# Autodesk Inventor assembly: HbSocketU02
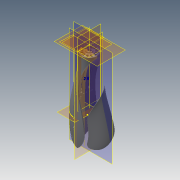
[picture p0: Inventor's stored thumbnail of the model, 180x180]
Saved by Autodesk Inventor 2015 SP1 (Build 190203100, 203)
## iProperties
Created: 2015-02-09
Part Number: HbSocketU02
Document SubType Name: Assembly
Designer: Yamaura
Author: Yamaura
## Documents named in this file (17)
- C:\Users\Yamaura\Documents\GitHub\HACKberry\HACKberry-hardware\3D\Inventor\Parts\HbSocketU02.iam
- C:\Users\Yamaura\Documents\GitHub\HACKberry\HACKberry-hardware\3D\Inventor\Parts\HbBatteryDoor03.ipt
- C:\Users\Yamaura\Documents\GitHub\HACKberry\HACKberry-hardware\3D\Inventor\Parts\HbBatteryDoorKnob03.ipt
- C:\Users\Yamaura\Documents\GitHub\HACKberry\HACKberry-hardware\3D\Inventor\Parts\HbBatteryHingeA03.ipt
- C:\Users\Yamaura\Documents\GitHub\HACKberry\HACKberry-hardware\3D\Inventor\Parts\HbBatteryHingeB03.ipt
- C:\Users\Yamaura\Documents\GitHub\HACKberry\HACKberry-hardware\3D\Inventor\Parts\HbBatteryHingeC03.ipt
- C:\Users\Yamaura\Documents\GitHub\HACKberry\HACKberry-hardware\3D\Inventor\Parts\HbBatteryCase01.ipt
- C:\Users\Yamaura\Documents\GitHub\HACKberry\HACKberry-hardware\3D\Inventor\Parts\HbBatteryLockKnob01.ipt
- C:\Users\Yamaura\Documents\GitHub\HACKberry\HACKberry-hardware\3D\Inventor\Parts\HbBatteryPcb01.ipt
- C:\Users\Yamaura\Documents\GitHub\HACKberry\HACKberry-hardware\3D\Inventor\Parts\DMW-BLF19.ipt
- C:\Users\Yamaura\Documents\GitHub\HACKberry\HACKberry-hardware\3D\Inventor\Parts\HbBatteryDoorLever03.ipt
- C:\Users\Yamaura\Documents\GitHub\HACKberry\HACKberry-hardware\3D\Inventor\Parts\HbMainFrameA01.ipt
- C:\Users\Yamaura\Documents\GitHub\HACKberry\HACKberry-hardware\3D\Inventor\Parts\HbMainFrameB01.ipt
- C:\Users\Yamaura\Documents\GitHub\HACKberry\HACKberry-hardware\3D\Inventor\Parts\HbUpperArmCover01.ipt
- C:\Users\Yamaura\Documents\GitHub\HACKberry\HACKberry-hardware\3D\Inventor\Parts\VN-3-1.ipt
- C:\Users\Yamaura\Documents\GitHub\HACKberry\HACKberry-hardware\3D\Inventor\Parts\TS 0.4-3.2-14.ipt
- C:\Users\Yamaura\Documents\GitHub\HACKberry\HACKberry-hardware\3D\Inventor\Parts\flatScrewM2L6PHI3.3T1.3.ipt
## Components (23 placed, 16 different names)
1. HbBatteryCase01:1 — メイト:29, メイト:30, メイト:34, メイト:35, メイト:36, フラッシュ:10, フラッシュ:11, フラッシュ:12, フラッシュ:13
2. HbBatteryLockKnob01:1 — メイト:30
3. HbBatteryPcb01:1 — メイト:29, メイト:61, メイト:62, メイト:63, メイト:64, メイト:69
4. DMW-BLF19:1 — メイト:34, メイト:35, メイト:36
5. flatScrewM2L6PHI3.3T1.3:1 — メイト:69, フラッシュ:10
6. flatScrewM2L6PHI3.3T1.3:2 — メイト:70, フラッシュ:12
7. flatScrewM2L6PHI3.3T1.3:3 — メイト:71, フラッシュ:13
8. flatScrewM2L6PHI3.3T1.3:4 — メイト:72, フラッシュ:11
9. TS 0.4-3.2-14:1 — メイト:73, 正接:1, 正接:2, 正接:3
10. VN-3-1:2 — メイト:62, メイト:63
11. HbBatteryHingeC03:1 — メイト:49, メイト:50, メイト:51
12. HbBatteryHingeB03:1 — メイト:40, メイト:45, メイト:47
13. HbBatteryHingeA03:1 — メイト:44, メイト:46
14. HbBatteryDoor03:1 — フラッシュ:5, メイト:44, メイト:45, メイト:46, メイト:47, メイト:49, メイト:50, メイト:51, 角度:3
15. HbMainFrameA01:1 — フラッシュ:6, フラッシュ:7, フラッシュ:8, メイト:52, メイト:53, メイト:54, メイト:73, 正接:1, 正接:2
16. VN-3-1:1 — メイト:61, メイト:64
17. HbBatteryDoorKnob03:3 — メイト:58, メイト:59, メイト:60, 正接:3
18. HbUpperArmCover01:1 — メイト:55, フラッシュ:9
19. HbMainFrameB01:1 — メイト:52, メイト:53, メイト:54, メイト:70, メイト:71, メイト:72
20. HbBatteryDoorKnob03:1 — メイト:37, メイト:38, メイト:39
21. HbBatteryDoorKnob03:2
22. HbBatteryDoorLever03:1 — メイト:37, メイト:38, メイト:39, メイト:58, メイト:59, メイト:60
23. HbBatteryDoorLever03:2
## Component patterns: (2 elements, first: HbBatteryDoorKnob03:1), (2 elements, first: HbBatteryDoorLever03:1)
## Relationships (45: Mate 32, Flush 9, Tangent 3, Angle 1)
- メイト:29 [Mate]: HbBatteryCase01:1 ↔ HbBatteryPcb01:1
- メイト:30 [Mate]: HbBatteryCase01:1 ↔ HbBatteryLockKnob01:1
- メイト:34 [Mate]: HbBatteryCase01:1 ↔ DMW-BLF19:1
- メイト:35 [Mate]: HbBatteryCase01:1 ↔ DMW-BLF19:1
- メイト:36 [Mate] (0.1 mm): HbBatteryCase01:1 ↔ DMW-BLF19:1
- メイト:37 [Mate]: HbBatteryDoorKnob03:1 ↔ HbBatteryDoorLever03:1
- メイト:38 [Mate]: HbBatteryDoorKnob03:1 ↔ HbBatteryDoorLever03:1
- メイト:39 [Mate]: HbBatteryDoorKnob03:1 ↔ HbBatteryDoorLever03:1
- メイト:40 [Mate]: HbBatteryHingeB03:1
- フラッシュ:5 [Flush]: HbBatteryDoor03:1
- メイト:44 [Mate]: HbBatteryHingeA03:1 ↔ HbBatteryDoor03:1
- メイト:45 [Mate]: HbBatteryHingeB03:1 ↔ HbBatteryDoor03:1
- メイト:46 [Mate]: HbBatteryHingeA03:1 ↔ HbBatteryDoor03:1
- メイト:47 [Mate]: HbBatteryHingeB03:1 ↔ HbBatteryDoor03:1
- メイト:49 [Mate]: HbBatteryHingeC03:1 ↔ HbBatteryDoor03:1
- メイト:50 [Mate]: HbBatteryHingeC03:1 ↔ HbBatteryDoor03:1
- メイト:51 [Mate]: HbBatteryHingeC03:1 ↔ HbBatteryDoor03:1
- 角度:3 [Angle] (0 deg): HbBatteryDoor03:1
- フラッシュ:6 [Flush] (-0.2 mm): HbMainFrameA01:1
- フラッシュ:7 [Flush]: HbMainFrameA01:1
- フラッシュ:8 [Flush]: HbMainFrameA01:1
- メイト:52 [Mate]: HbMainFrameA01:1 ↔ HbMainFrameB01:1
- メイト:53 [Mate]: HbMainFrameA01:1 ↔ HbMainFrameB01:1
- メイト:54 [Mate] (0.2 mm): HbMainFrameA01:1 ↔ HbMainFrameB01:1
- メイト:55 [Mate]: HbUpperArmCover01:1
- フラッシュ:9 [Flush]: HbUpperArmCover01:1
- メイト:58 [Mate]: HbBatteryDoorKnob03:3 ↔ HbBatteryDoorLever03:1
- メイト:59 [Mate]: HbBatteryDoorKnob03:3 ↔ HbBatteryDoorLever03:1
- メイト:60 [Mate]: HbBatteryDoorKnob03:3 ↔ HbBatteryDoorLever03:1
- メイト:61 [Mate]: HbBatteryPcb01:1 ↔ VN-3-1:1
- メイト:62 [Mate]: HbBatteryPcb01:1 ↔ VN-3-1:2
- メイト:63 [Mate]: HbBatteryPcb01:1 ↔ VN-3-1:2
- メイト:64 [Mate]: HbBatteryPcb01:1 ↔ VN-3-1:1
- メイト:69 [Mate]: HbBatteryPcb01:1 ↔ flatScrewM2L6PHI3.3T1.3:1
- フラッシュ:10 [Flush]: HbBatteryCase01:1 ↔ flatScrewM2L6PHI3.3T1.3:1
- メイト:70 [Mate]: flatScrewM2L6PHI3.3T1.3:2 ↔ HbMainFrameB01:1
- メイト:71 [Mate]: flatScrewM2L6PHI3.3T1.3:3 ↔ HbMainFrameB01:1
- メイト:72 [Mate]: flatScrewM2L6PHI3.3T1.3:4 ↔ HbMainFrameB01:1
- フラッシュ:11 [Flush]: HbBatteryCase01:1 ↔ flatScrewM2L6PHI3.3T1.3:4
- フラッシュ:12 [Flush]: HbBatteryCase01:1 ↔ flatScrewM2L6PHI3.3T1.3:2
- フラッシュ:13 [Flush]: HbBatteryCase01:1 ↔ flatScrewM2L6PHI3.3T1.3:3
- メイト:73 [Mate] (-2.4 mm): TS 0.4-3.2-14:1 ↔ HbMainFrameA01:1
- 正接:1 [Tangent]: TS 0.4-3.2-14:1 ↔ HbMainFrameA01:1
- 正接:2 [Tangent]: TS 0.4-3.2-14:1 ↔ HbMainFrameA01:1
- 正接:3 [Tangent]: TS 0.4-3.2-14:1 ↔ HbBatteryDoorKnob03:3
